# Autodesk Inventor assembly: layer2
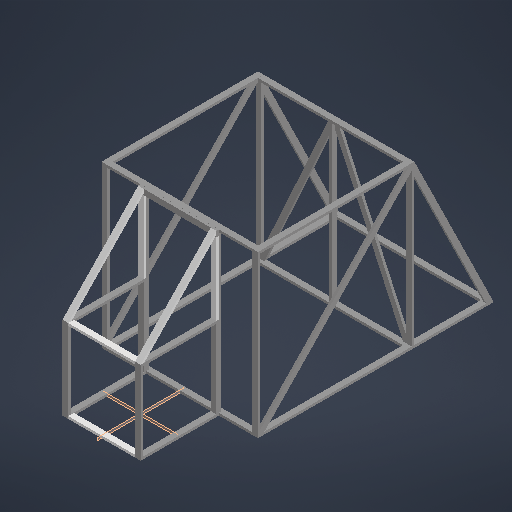
[picture p0: Inventor's stored thumbnail of the model, 512x512]
Saved by Autodesk Inventor 2026 (Build 300175000, 175)
## iProperties
Created: 2024-09-19
Part Number: layer2
Document SubType Name: Assembly
Designer: User
Author: User
## Documents named in this file (18)
- C:\Users\trott\Documents\UofSC-ASME-Tiger-Burn-Design-2025\CAD\Body\Base 03\Base 03.iam
- C:\Users\trott\Documents\UofSC-ASME-Tiger-Burn-Design-2025\CAD\Body\Base 03\12'x2x4.ipt
- C:\Users\trott\Documents\UofSC-ASME-Tiger-Burn-Design-2025\CAD\Body\Base 03\7'5x2x4.ipt
- C:\Users\trott\Documents\UofSC-ASME-Tiger-Burn-Design-2025\CAD\Body\Base 03\8'x2x4.ipt
- C:\Users\trott\Documents\UofSC-ASME-Tiger-Burn-Design-2025\CAD\Body\Base 03\s48x2x4b.ipt
- C:\Users\trott\Documents\UofSC-ASME-Tiger-Burn-Design-2025\CAD\Body\Base 03\s88x2x4.ipt
- C:\Users\trott\Documents\UofSC-ASME-Tiger-Burn-Design-2025\CAD\Body\Base 03\s48x2x4a.ipt
- C:\Users\trott\Documents\UofSC-ASME-Tiger-Burn-Design-2025\CAD\Reference (TB24)\F_Legs2\4x2x4.ipt
- C:\Users\trott\Documents\UofSC-ASME-Tiger-Burn-Design-2025\CAD\Body\Base 03\2x4x41.ipt
- C:\Users\trott\Documents\UofSC-ASME-Tiger-Burn-Design-2025\CAD\Reference (TB24)\F_Legs2\4x2x4_MIR1.ipt
- C:\Users\trott\Documents\UofSC-ASME-Tiger-Burn-Design-2025\CAD\Reference (TB24)\F_Legs2\4x2x4_MIR2.ipt
- C:\Users\trott\Documents\UofSC-ASME-Tiger-Burn-Design-2025\CAD\Reference (TB24)\F_Legs2\4x2x4_MIR1_MIR.ipt
- C:\Users\trott\Documents\UofSC-ASME-Tiger-Burn-Design-2025\CAD\Body\Base 03\2x4x44.5.ipt
- C:\Users\trott\Documents\UofSC-ASME-Tiger-Burn-Design-2025\CAD\Body\Base 03\2x4x44.5_MIR.ipt
- C:\Users\trott\Documents\UofSC-ASME-Tiger-Burn-Design-2025\CAD\Body\Base 03\S_2x4x66.83.ipt
- C:\Users\trott\Documents\UofSC-ASME-Tiger-Burn-Design-2025\CAD\Body\Base 03\S_2x4x66.83_MIR.ipt
- C:\Users\trott\Documents\UofSC-ASME-Tiger-Burn-Design-2025\CAD\Body\Base 03\2x4x96.ipt
- C:\Users\trott\Documents\UofSC-ASME-Tiger-Burn-Design-2025\CAD\Body\Base 03\2x4x96_MIR.ipt
## Components (37 placed, 17 different names)
1. 12'x2x4:1 — Flush:3, Flush:4, Flush:5, Mate:2, Mate:3, Mate:5, Flush:15, Flush:16, Flush:17, Flush:38, Flush:41
2. 12'x2x4:2 — Flush:3, Flush:4, Flush:5, Mate:1, Flush:6, Flush:7, Flush:8, Flush:9, Flush:10, Mate:4, Mate:6, Flush:12, Flush:13, Flush:14, Mate:24, Flush:43
3. 7'5x2x4:1 — Mate:1, Flush:6, Flush:7, Flush:11, Mate:25, Flush:40, Mate:26, Flush:42
4. 7'5x2x4:2 — Flush:10, Flush:11, Flush:18, Flush:19, Mate:11, Flush:28
5. 7'5x2x4:3 — Flush:8, Flush:9, Mate:2
6. 8'x2x4:1 — Mate:4, Flush:13, Flush:14, Mate:8, Flush:21, Flush:22, Flush:36
7. 8'x2x4:2 — Mate:3, Flush:15, Flush:16, Mate:7, Flush:20, Flush:23
8. 8'x2x4:3 — Mate:5, Flush:17, Flush:18, Flush:31, Mate:22
9. 8'x2x4:4 — Mate:6, Flush:12, Flush:19, Mate:23, Flush:39
10. 8'x2x4:5 — Mate:8, Flush:21, Flush:22, Mate:9, Flush:26, Mate:10, Flush:27
11. 8'x2x4:6 — Mate:7, Flush:20, Flush:23, Flush:24, Flush:25, Mate:21, Flush:37
12. 7'5x2x4:4 — Flush:24, Mate:10, Flush:27, Mate:35, Flush:63
13. 7'5x2x4:5 — Flush:25, Mate:9, Flush:26, Mate:18, Mate:20
14. 8'x2x4:8 — Mate:11, Flush:28, Flush:31, Mate:17, Flush:34, Mate:19, Flush:35
15. s48x2x4b:3 — Mate:17, Mate:18, Flush:34
16. s48x2x4b:4 — Mate:19, Mate:20, Flush:35
17. s88x2x4:1 — Flush:36
18. s88x2x4:2 — Mate:21, Mate:22, Flush:37
19. s48x2x4a:1 — Flush:38
20. s48x2x4a:2 — Mate:23, Mate:24, Flush:39
21. 4x2x4:1 — Mate:25, Flush:40, Flush:41, Flush:44, Flush:46, Mate:28, Flush:47, Flush:48
22. 4x2x4:2 — Mate:26, Flush:42, Flush:43, Mate:27, Flush:45, Flush:49
23. 2x4x41:1 — Flush:44, Mate:27, Flush:45, Flush:56
24. 4x2x4:3 — Flush:46, Mate:28, Flush:47, Flush:48, Flush:52, Mate:30, Flush:53
25. 4x2x4_MIR1:1 — Mate:29, Flush:50, Flush:51
26. 4x2x4:4 — Mate:29, Flush:50, Flush:51, Flush:54, Mate:31, Flush:55, Mate:32, Flush:57
27. 4x2x4:5 — Flush:52, Mate:30, Flush:53
28. 2x4x41:2 — Flush:54, Mate:31, Flush:55
29. 4x2x4_MIR2:1
30. 4x2x4_MIR1_MIR:1 — Flush:58
31. 2x4x44.5:1 — Mate:32, Flush:57, Flush:58, Flush:59, Mate:33, Flush:60, Flush:61, Flush:62
32. 4x2x4:6 — Flush:59, Mate:33, Flush:60, Mate:34
33. 2x4x44.5_MIR:1
34. S_2x4x66.83:1 — Mate:34, Flush:61
35. S_2x4x66.83_MIR:1
36. 2x4x96:1 — Mate:35, Flush:62, Flush:63
37. 2x4x96_MIR:1
## Relationships (87: Flush 57, Mate 30)
- Flush:3 (2349.5 mm): 12'x2x4:1 ↔ 12'x2x4:2
- Flush:4: 12'x2x4:1 ↔ 12'x2x4:2
- Flush:5: 12'x2x4:1 ↔ 12'x2x4:2
- Mate:1: 12'x2x4:2 ↔ 7'5x2x4:1
- Flush:6: 12'x2x4:2 ↔ 7'5x2x4:1
- Flush:7: 12'x2x4:2 ↔ 7'5x2x4:1
- Flush:8: 12'x2x4:2 ↔ 7'5x2x4:3
- Flush:9: 12'x2x4:2 ↔ 7'5x2x4:3
- Mate:2: 12'x2x4:1 ↔ 7'5x2x4:3
- Flush:10: 12'x2x4:2 ↔ 7'5x2x4:2
- Flush:11 (2349.5 mm): 7'5x2x4:1 ↔ 7'5x2x4:2
- Mate:3: 12'x2x4:1 ↔ 8'x2x4:2
- Mate:4: 12'x2x4:2 ↔ 8'x2x4:1
- Mate:5: 12'x2x4:1 ↔ 8'x2x4:3
- Mate:6: 12'x2x4:2 ↔ 8'x2x4:4
- Flush:12: 12'x2x4:2 ↔ 8'x2x4:4
- Flush:13: 12'x2x4:2 ↔ 8'x2x4:1
- Flush:14: 12'x2x4:2 ↔ 8'x2x4:1
- Flush:15: 12'x2x4:1 ↔ 8'x2x4:2
- Flush:16: 12'x2x4:1 ↔ 8'x2x4:2
- Flush:17: 12'x2x4:1 ↔ 8'x2x4:3
- Flush:18: 7'5x2x4:2 ↔ 8'x2x4:3
- Flush:19: 7'5x2x4:2 ↔ 8'x2x4:4
- Mate:7: 8'x2x4:2 ↔ 8'x2x4:6
- Mate:8: 8'x2x4:1 ↔ 8'x2x4:5
- Flush:20: 8'x2x4:2 ↔ 8'x2x4:6
- Flush:21: 8'x2x4:1 ↔ 8'x2x4:5
- Flush:22: 8'x2x4:1 ↔ 8'x2x4:5
- Flush:23: 8'x2x4:2 ↔ 8'x2x4:6
- Flush:24: 8'x2x4:6 ↔ 7'5x2x4:4
- Flush:25: 8'x2x4:6 ↔ 7'5x2x4:5
- Mate:9: 8'x2x4:5 ↔ 7'5x2x4:5
- Flush:26: 8'x2x4:5 ↔ 7'5x2x4:5
- Mate:10: 8'x2x4:5 ↔ 7'5x2x4:4
- Flush:27: 8'x2x4:5 ↔ 7'5x2x4:4
- Mate:11: 7'5x2x4:2 ↔ 8'x2x4:8
- Flush:28: 7'5x2x4:2 ↔ 8'x2x4:8
- Flush:31 (1200.15 mm): 8'x2x4:3 ↔ 8'x2x4:8
- Mate:17: 8'x2x4:8 ↔ s48x2x4b:3
- Mate:18: 7'5x2x4:5 ↔ s48x2x4b:3
- Flush:34: 8'x2x4:8 ↔ s48x2x4b:3
- Mate:19: 8'x2x4:8 ↔ s48x2x4b:4
- Mate:20: 7'5x2x4:5 ↔ s48x2x4b:4
- Flush:35: 8'x2x4:8 ↔ s48x2x4b:4
- Flush:36: 8'x2x4:1 ↔ s88x2x4:1
- Mate:21: 8'x2x4:6 ↔ s88x2x4:2
- Mate:22: 8'x2x4:3 ↔ s88x2x4:2
- Flush:37: 8'x2x4:6 ↔ s88x2x4:2
- Flush:38: 12'x2x4:1 ↔ s48x2x4a:1
- Mate:23: 8'x2x4:4 ↔ s48x2x4a:2
- Mate:24: 12'x2x4:2 ↔ s48x2x4a:2
- Flush:39: 8'x2x4:4 ↔ s48x2x4a:2
- Mate:25: 7'5x2x4:1 ↔ 4x2x4:1
- Flush:40: 7'5x2x4:1 ↔ 4x2x4:1
- Flush:41 (609.6 mm): 12'x2x4:1 ↔ 4x2x4:1
- Mate:26: 7'5x2x4:1 ↔ 4x2x4:2
- Flush:42: 7'5x2x4:1 ↔ 4x2x4:2
- Flush:43 (609.6 mm): 12'x2x4:2 ↔ 4x2x4:2
- Flush:44: 4x2x4:1 ↔ 2x4x41:1
- Mate:27: 4x2x4:2 ↔ 2x4x41:1
- Flush:45: 4x2x4:2 ↔ 2x4x41:1
- Flush:46: 4x2x4:1 ↔ 4x2x4:3
- Mate:28: 4x2x4:1 ↔ 4x2x4:3
- Flush:47: 4x2x4:1 ↔ 4x2x4:3
- Flush:48: 4x2x4:1 ↔ 4x2x4:3
- Flush:49 (-609.6 mm): 4x2x4:2
- Mate:29: 4x2x4_MIR1:1 ↔ 4x2x4:4
- Flush:50: 4x2x4_MIR1:1 ↔ 4x2x4:4
- Flush:51: 4x2x4_MIR1:1 ↔ 4x2x4:4
- Flush:52: 4x2x4:3 ↔ 4x2x4:5
- Mate:30: 4x2x4:3 ↔ 4x2x4:5
- Flush:53: 4x2x4:3 ↔ 4x2x4:5
- Flush:54: 4x2x4:4 ↔ 2x4x41:2
- Mate:31: 4x2x4:4 ↔ 2x4x41:2
- Flush:55: 4x2x4:4 ↔ 2x4x41:2
- Flush:56 (-609.6 mm): 2x4x41:1
- Mate:32: 4x2x4:4 ↔ 2x4x44.5:1
- Flush:57: 4x2x4:4 ↔ 2x4x44.5:1
- Flush:58: 4x2x4_MIR1_MIR:1 ↔ 2x4x44.5:1
- Flush:59: 2x4x44.5:1 ↔ 4x2x4:6
- Mate:33: 2x4x44.5:1 ↔ 4x2x4:6
- Flush:60: 2x4x44.5:1 ↔ 4x2x4:6
- Mate:34: 4x2x4:6 ↔ S_2x4x66.83:1
- Flush:61: 2x4x44.5:1 ↔ S_2x4x66.83:1
- Mate:35: 7'5x2x4:4 ↔ 2x4x96:1
- Flush:62: 2x4x44.5:1 ↔ 2x4x96:1
- Flush:63: 7'5x2x4:4 ↔ 2x4x96:1
